# Autodesk Inventor assembly: Assignment 5
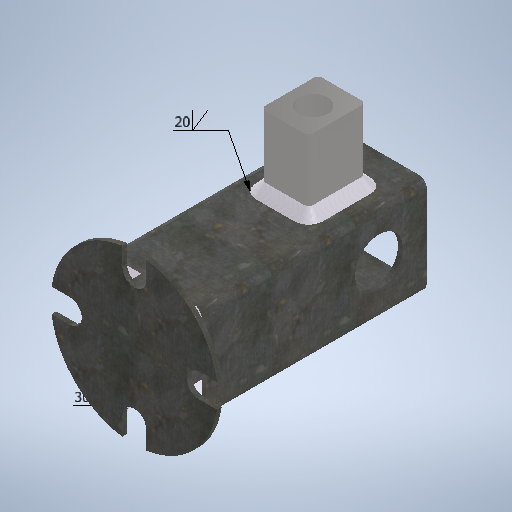
[picture p0: Inventor's stored thumbnail of the model, 512x512]
Saved by Autodesk Inventor 2025.2 (Build 292293000, 293)
## iProperties
Created: 2025-04-01
Part Number: Assignment 5
Document SubType Name: Weldment
Designer: bless
Weld Material: Welded Aluminum-6061
Author: bless
## Documents named in this file (4)
- C:\Users\bless\OneDrive - Conestoga College\Documents\Inventor\8071W25\weldmants\Assignment 5 Blesson\Assignment 5.iam
- C:\Users\bless\OneDrive - Conestoga College\Documents\Inventor\8071W25\weldmants\Assignment 5 Blesson\Base.ipt
- C:\Users\bless\OneDrive - Conestoga College\Documents\Inventor\8071W25\weldmants\Assignment 5 Blesson\Central.ipt
- C:\Users\bless\OneDrive - Conestoga College\Documents\Inventor\8071W25\weldmants\Assignment 5 Blesson\cantiliever.ipt
## Components (3 placed, 3 different names)
1. Base:1 — Flush:1
2. Central:1 — Flush:1, Flush:2
3. cantiliever:1 — Flush:2
## Relationships (2: Flush 2)
- Flush:1: Base:1 ↔ Central:1
- Flush:2: Central:1 ↔ cantiliever:1
